# Autodesk Inventor assembly: Assembly2 22
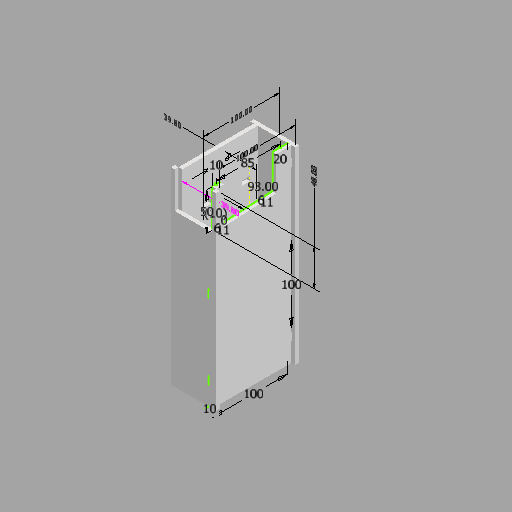
[picture p0: Inventor's stored thumbnail of the model, 512x512]
Saved by Autodesk Inventor 2025.3 (Build 293356000, 356)
## iProperties
Created: 2026-04-06
Part Number: Assembly2 22
Document SubType Name: Assembly
Designer: user
Author: user
## Documents named in this file (5)
- C:\Ayman\Inventor Projects\Lifting Mechanism\Assembly2 22.iam
- C:\Ayman\Inventor Projects\Lifting Mechanism\Lifting Sections left.ipt
- C:\Ayman\Inventor Projects\Lifting Mechanism\Lifting Sections leftt.ipt
- C:\Ayman\Inventor Projects\Lifting Mechanism\Lifting Sections right.ipt
- C:\Ayman\Inventor Projects\Lifting Mechanism\Lifting Sections back.ipt
## Components (4 placed, 4 different names)
1. Lifting Sections left:1 — Mate:3, Mate:4, Flush:2, Flush:3, Mate:5, Mate:6
2. Lifting Sections leftt:1 — Flush:1, Mate:1, Mate:2, Mate:3, Mate:4, Flush:2
3. Lifting Sections right:1 — Flush:1, Mate:1, Mate:2
4. Lifting Sections back:1 — Flush:3, Mate:5, Mate:6
## Relationships (9: Mate 6, Flush 3)
- Flush:1: Lifting Sections leftt:1 ↔ Lifting Sections right:1
- Mate:1: Lifting Sections leftt:1 ↔ Lifting Sections right:1
- Mate:2: Lifting Sections leftt:1 ↔ Lifting Sections right:1
- Mate:3: Lifting Sections left:1 ↔ Lifting Sections leftt:1
- Mate:4: Lifting Sections left:1 ↔ Lifting Sections leftt:1
- Flush:2: Lifting Sections left:1 ↔ Lifting Sections leftt:1
- Flush:3: Lifting Sections left:1 ↔ Lifting Sections back:1
- Mate:5: Lifting Sections left:1 ↔ Lifting Sections back:1
- Mate:6: Lifting Sections left:1 ↔ Lifting Sections back:1
